# Autodesk Inventor assembly: Roll_Fixation_Frame_8mm_Set
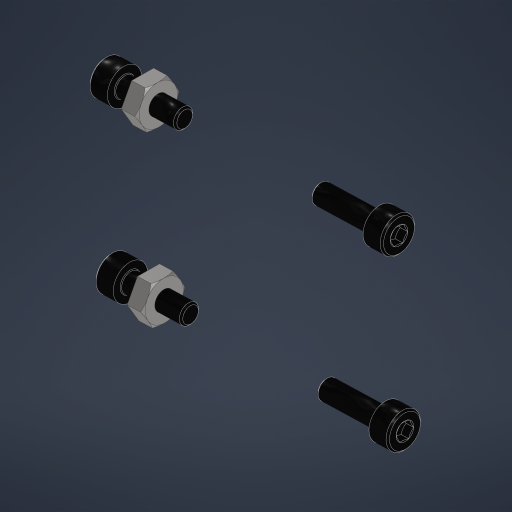
[picture p0: Inventor's stored thumbnail of the model, 512x512]
Saved by Autodesk Inventor 2024 (Build 280153000, 153)
## iProperties
Created: 2024-01-28
Part Number: Roll_Fixation_Frame_8mm_Set
Document SubType Name: Assembly
Designer: 김대겸
Author: 김대겸
## Documents named in this file (3)
- C:\Users\김대겸\Desktop\2024_Robit_Hardware\ROBOCUP_2024_eindhoven\부품\Bolt_Washer_Nut\Roll_Fixation_Frame_8mm_Set.iam
- C:\Users\김대겸\Desktop\2024_Robit_Hardware\ROBOCUP_2024_eindhoven\부품\Bolt_Washer_Nut\CSH-ST-M2_5-8_203.ipt
- C:\Users\김대겸\Desktop\2024_Robit_Hardware\ROBOCUP_2024_eindhoven\부품\Bolt_Washer_Nut\SLBNR2_5.ipt
## Components (6 placed, 2 different names)
1. CSH-ST-M2_5-8_203:1
2. CSH-ST-M2_5-8_203:2
3. SLBNR2_5:1
4. CSH-ST-M2_5-8_203:3
5. SLBNR2_5:2
6. CSH-ST-M2_5-8_203:4
## Relationships (4: Flush 2, Mate 2)
- [Flush]: CSH-ST-M2_5-8_203:3 ↔ CSH-ST-M2_5-8_203:4
- [Flush]: CSH-ST-M2_5-8_203:1 ↔ CSH-ST-M2_5-8_203:2
- [Mate]: SLBNR2_5:2 ↔ CSH-ST-M2_5-8_203:4
- [Mate]: SLBNR2_5:1 ↔ CSH-ST-M2_5-8_203:3
